# Autodesk Inventor assembly: 54132-GE02_tapa
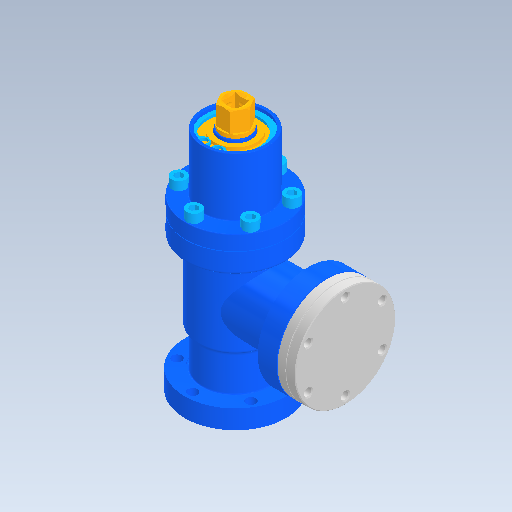
[picture p0: Inventor's stored thumbnail of the model, 512x512]
Saved by Autodesk Inventor 2020 (Build 240168000, 168)
## iProperties
Created: 2014-04-14
Part Number: 54132-GE02_tapa
Document SubType Name: Assembly
Designer: General
Sending System: SIEMENS PLM Software NX 7.5
Preprocessor: ST-DEVELOPER v11
Title: 1087050739_203.stp
## Documents named in this file (11)
- C:\LAFriOC\diseños\sistema de vacío\Componentes Sistema de vacio\54132-GE02_tapa.iam
- C:\Users\General\Downloads\475901.ipt
- C:\Users\General\Downloads\218189.ipt
- C:\Users\General\Downloads\475865.ipt
- C:\Users\General\Downloads\475872.ipt
- C:\Users\General\Downloads\491522.ipt
- C:\Users\General\Downloads\N-6203-440.1.ipt
- C:\Users\General\Downloads\222101_2.ipt
- C:\Users\General\Downloads\257611.ipt
- C:\Users\General\Downloads\432708.iam
- C:\LAFriOC\diseños\sistema de vacío\Componentes Sistema de vacio\blankf0275x000nm.ipt
## Components (17 placed, 17 different names)
1. 475901_1003
2. 218189_1004
3. 218189_1005
4. 218189_1006
5. 218189_1007
6. 218189_1008
7. 218189_1009
8. 475865_1010
9. 475872_1011
10. 491522_1012
11. N-6203-440.1_1013
12. 222101_2_1014
13. 257611_1015
14. 222101_2_1016
15. 257611_1017 — De rotación:1
16. 432708_1018 [sub-assembly]
17. blankf0275x000nm:1 — De rotación:1
## Relationships (1: RevoluteJoint 1)
- De rotación:1 [RevoluteJoint]: 257611_1017 ↔ blankf0275x000nm:1
